# Autodesk Inventor assembly: Cup_Dispenser
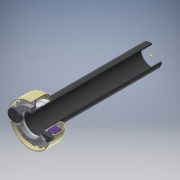
[picture p0: Inventor's stored thumbnail of the model, 180x180]
Saved by Autodesk Inventor 2016 (Build 200138000, 138)
## iProperties
Created: 2015-07-19
Part Number: Cup_Dispenser
Document SubType Name: Assembly
Designer: bastli
Author: bastli
## Documents named in this file (7)
- C:\Users\3DPrinterUser\Documents\GitHub\BarBot\Conception\Mechanical\Cup_Dispenser_3\Cup_Dispenser.iam
- C:\Users\3DPrinterUser\Documents\GitHub\BarBot\Conception\Mechanical\Cup_Dispenser_3\Fixture.ipt
- C:\Users\3DPrinterUser\Documents\GitHub\BarBot\Conception\Mechanical\Cup_Dispenser_3\Transmission.ipt
- C:\Users\3DPrinterUser\Documents\GitHub\BarBot\Conception\Mechanical\Cup_Dispenser_3\Nema 8.ipt
- C:\Users\3DPrinterUser\Documents\GitHub\BarBot\Conception\Mechanical\Cup_Dispenser_3\Funnel_Adapter.ipt
- C:\Users\3DPrinterUser\Documents\GitHub\BarBot\Conception\Mechanical\Cup_Dispenser_3\Hull.ipt
- C:\Users\3DPrinterUser\Documents\GitHub\BarBot\Conception\Mechanical\Cup_Dispenser\Cup_Dispenser_Pipe.ipt
## Components (9 placed, 6 different names)
1. Fixture:1 — Rigid:1, Rigid:3, Flush:1, Rotational:3, Flush:2, Rigid:4
2. Transmission:1 — Rotational:1
3. Nema 8:1 — Rigid:1, Rotational:1
4. Nema 8:2 — Rigid:3, Rotational:2
5. Transmission:2 — Rotational:2
6. Funnel_Adapter:1 — Flush:1
7. Funnel_Adapter:2 — Rotational:3
8. Hull:1 — Flush:2
9. Cup_Dispenser_Pipe:1 — Rigid:4
## Relationships (8: WeldJoint 3, RevoluteJoint 3, Flush 2)
- Rigid:1 [WeldJoint]: Fixture:1 ↔ Nema 8:1
- Rotational:1 [RevoluteJoint]: Transmission:1 ↔ Nema 8:1
- Rigid:3 [WeldJoint]: Fixture:1 ↔ Nema 8:2
- Rotational:2 [RevoluteJoint]: Nema 8:2 ↔ Transmission:2
- Flush:1: Fixture:1 ↔ Funnel_Adapter:1
- Rotational:3 [RevoluteJoint]: Fixture:1 ↔ Funnel_Adapter:2
- Flush:2: Fixture:1 ↔ Hull:1
- Rigid:4 [WeldJoint]: Fixture:1 ↔ Cup_Dispenser_Pipe:1
